# Autodesk Inventor assembly: UpperLevel
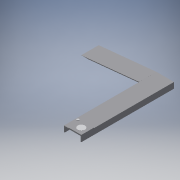
[picture p0: Inventor's stored thumbnail of the model, 180x180]
Saved by Autodesk Inventor 2019 (Build 230136000, 136)
## iProperties
Created: 2018-09-21
Part Number: UpperLevel
Document SubType Name: Assembly
Designer: user
Author: user
## Documents named in this file (7)
- C:\Users\user\Desktop\Roombotics\UpperLevel.iam
- C:\Users\user\Desktop\Roombotics\Side1.ipt
- C:\Users\user\Desktop\Roombotics\Top.ipt
- C:\Users\user\Desktop\Roombotics\Ramp1.ipt
- C:\Users\user\Desktop\Roombotics\Stove.ipt
- C:\Users\user\Desktop\Roombotics\Button.ipt
- C:\Users\user\Desktop\Roombotics\Burner.ipt
## Components (7 placed, 6 different names)
1. Side1:1 — Flush:1
2. Top:1 — Flush:1, Rigid:1, Flush:2, Flush:3, Flush:4
3. Side1:2 — Rigid:1
4. Ramp1:1 — Flush:2
5. Stove:1 — Flush:3, Flush:5
6. Button:1 — Flush:4
7. Burner:1 — Flush:5
## Relationships (6: Flush 5, WeldJoint 1)
- Flush:1: Side1:1 ↔ Top:1
- Rigid:1 [WeldJoint]: Top:1 ↔ Side1:2
- Flush:2: Top:1 ↔ Ramp1:1
- Flush:3: Top:1 ↔ Stove:1
- Flush:4: Top:1 ↔ Button:1
- Flush:5: Stove:1 ↔ Burner:1
